# Autodesk Inventor assembly: Assem1
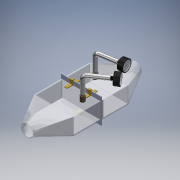
[picture p0: Inventor's stored thumbnail of the model, 180x180]
Saved by Autodesk Inventor 2017 (Build 210142000, 142)
## iProperties
Created: 2014-08-02
Part Number: Assem1
Document SubType Name: Assembly
Designer: XuZhiqing
Sending System: SolidWorks 2014
Last Author: 1
Last Saved: 2014-09-23
Author: XuZhiqing
## Documents named in this file (4)
- C:\Users\XuZhiqing\Desktop\Project01-CFD_the_sys\CAD-Whole Sys\filter and gauge\filter and gauge\filter and gauge.iam
- C:\Users\XuZhiqing\Desktop\Project01-CFD_the_sys\CAD-Whole Sys\filter and gauge\filter and gauge\Solid9.ipt
- C:\Users\XuZhiqing\Desktop\Project01-CFD_the_sys\CAD-Whole Sys\filter and gauge\filter\Assem1.iam
- C:\Users\XuZhiqing\Desktop\Project01-CFD_the_sys\CAD-Whole Sys\filter and gauge\filter and gauge\pressure gauge.iam
## Components (4 placed, 3 different names)
1. Solid9:1
2. Assem1:1 [sub-assembly] — Mate:1, Mate:2
3. pressure gauge:1 [sub-assembly] — Mate:1
4. pressure gauge:2 [sub-assembly] — Mate:2
## Relationships (2: Mate 2)
- Mate:1: Assem1:1 ↔ pressure gauge:1
- Mate:2: Assem1:1 ↔ pressure gauge:2
